# Autodesk Inventor assembly: ArmBase
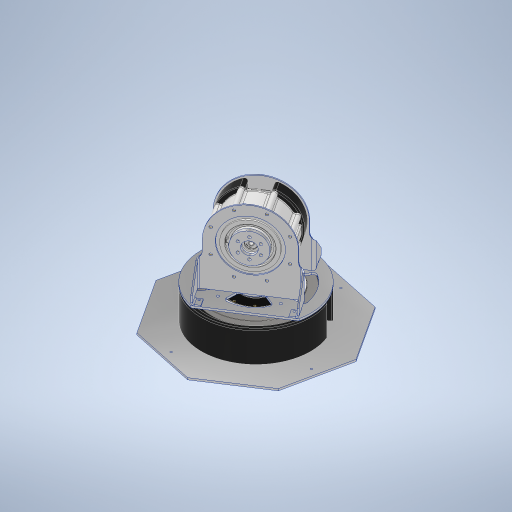
[picture p0: Inventor's stored thumbnail of the model, 512x512]
Saved by Autodesk Inventor 2024.3 (Build 283343010, 343A)
## iProperties
Created: 2025-05-20
Part Number: ArmBase
Document SubType Name: Assembly
Designer: kshau
Mass: 3061.84 g
Surface Area: 4858.08 cm^2
Volume: 1053.88 cm^3
Density: 2.9053 g/cm^3
Author: kshau
## Documents named in this file (16)
- C:\Users\kshau\Documents\inventor\Create_ViperX\Create_ViperX_ALOHA\Base_Component\ArmBase.iam
- C:\Users\kshau\Documents\inventor\Create_ViperX\Create_ViperX_ALOHA\Base_Component\base_parameter.ipt
- C:\Users\kshau\Documents\inventor\Create_ViperX\Create_ViperX_ALOHA\Actuator\RS02\RS02\RS02.iam
- C:\Users\kshau\Documents\inventor\Create_ViperX\Create_ViperX_ALOHA\BasicParts\TurnTable\TurnTable_140\TurnTable_140.iam
- C:\Users\kshau\Documents\inventor\Create_ViperX\Create_ViperX_ALOHA\Actuator\RS03\RS03\RS03.iam
- C:\Users\kshau\Documents\inventor\Create_ViperX\Create_ViperX_ALOHA\Base_Component\basefixplate1_forR3.ipt
- C:\Users\kshau\Documents\inventor\Create_ViperX\Create_ViperX_ALOHA\Base_Component\basefixpart_forR3.ipt
- C:\Users\kshau\Documents\inventor\Create_ViperX\Create_ViperX_ALOHA\Base_Component\basefixplate2_forR3.ipt
- C:\Users\kshau\Documents\inventor\Create_ViperX\Create_ViperX_ALOHA\Base_Component\servoplate_forR3.ipt
- C:\Users\kshau\Documents\inventor\Create_ViperX\Create_ViperX_ALOHA\Base_Component\baseplate_R2toR3.ipt
- C:\Users\kshau\Documents\inventor\Create_ViperX\Create_ViperX_ALOHA\Base_Component\basepart1_forR2.ipt
- C:\Users\kshau\Documents\inventor\Create_ViperX\Create_ViperX_ALOHA\Base_Component\basepart2_forR2.ipt
- C:\Users\kshau\Documents\inventor\Create_ViperX\Create_ViperX_ALOHA\NessesaryParts\ALSBF10-40-M4-N4\ALSBF10-40-M4-N4\ALSBF10-40-M4-N4.ipt
- C:\Users\kshau\Documents\inventor\Create_ViperX\Create_ViperX_ALOHA\Base_Component\Largebaseplate.ipt
- C:\Users\kshau\Documents\inventor\Create_ViperX\Create_ViperX_ALOHA\BasicParts\Bearing\NMB_RF2210X2HH\RF-2210X2HH.iam
- C:\Users\kshau\Documents\inventor\Create_ViperX\Create_ViperX_ALOHA\Base_Component\basespacer1.ipt
## Components (19 placed, 15 different names)
1. base_parameter:1
2. RS02:1 [sub-assembly] — メイト:1, 回転:15, 回転:16, 回転:17, メイト:2, 回転:29
3. TurnTable_140:1 [sub-assembly] — メイト:1, 回転:18, 回転:19, 回転:20, 回転:21, 回転:27, 回転:28
4. RS03:1 [sub-assembly] — 回転:3, 回転:4, 回転:5, 回転:6, 回転:9, 回転:10
5. basefixplate1_forR3:1 — 回転:3, 回転:4, 回転:26, フラッシュ:3
6. basefixpart_forR3:1 — 回転:5, 回転:6, 回転:11, 回転:12, メイト:5, メイト:6
7. basefixplate2_forR3:1 — 回転:11, 回転:12, 回転:25, フラッシュ:4
8. servoplate_forR3:1 — 回転:9, 回転:10
9. baseplate_R2toR3:1 — 回転:15, 回転:25, 回転:26, フラッシュ:3, フラッシュ:4, 回転:29, 回転:30, 回転:31
10. basepart1_forR2:1 — 回転:16, 回転:17, フラッシュ:1, フラッシュ:2, メイト:4, 回転:24
11. basepart2_forR2:1 — フラッシュ:1, メイト:2, メイト:3
12. ALSBF10-40-M4-N4:1 — 回転:18
13. ALSBF10-40-M4-N4:2 — 回転:19
14. ALSBF10-40-M4-N4:3 — 回転:20, 回転:23
15. ALSBF10-40-M4-N4:4 — 回転:21, 回転:22
16. basepart2_forR2:2 — フラッシュ:2, メイト:3, メイト:4
17. Largebaseplate:1 — 回転:22, 回転:23, 回転:24
18. RF-2210X2HH:1 [sub-assembly] — メイト:5, メイト:6
19. basespacer1:1 — 回転:27, 回転:28, 回転:30, 回転:31
## Relationships (35: RevoluteJoint 25, Mate 6, Flush 4)
- メイト:1 [Mate]: RS02:1 ↔ TurnTable_140:1
- 回転:3 [RevoluteJoint]: RS03:1 ↔ basefixplate1_forR3:1
- 回転:4 [RevoluteJoint]: RS03:1 ↔ basefixplate1_forR3:1
- 回転:5 [RevoluteJoint]: RS03:1 ↔ basefixpart_forR3:1
- 回転:6 [RevoluteJoint]: RS03:1 ↔ basefixpart_forR3:1
- 回転:9 [RevoluteJoint]: RS03:1 ↔ servoplate_forR3:1
- 回転:10 [RevoluteJoint]: RS03:1 ↔ servoplate_forR3:1
- 回転:11 [RevoluteJoint]: basefixpart_forR3:1 ↔ basefixplate2_forR3:1
- 回転:12 [RevoluteJoint]: basefixpart_forR3:1 ↔ basefixplate2_forR3:1
- 回転:15 [RevoluteJoint]: RS02:1 ↔ baseplate_R2toR3:1
- 回転:16 [RevoluteJoint]: RS02:1 ↔ basepart1_forR2:1
- 回転:17 [RevoluteJoint]: RS02:1 ↔ basepart1_forR2:1
- 回転:18 [RevoluteJoint]: TurnTable_140:1 ↔ ALSBF10-40-M4-N4:1
- 回転:19 [RevoluteJoint]: TurnTable_140:1 ↔ ALSBF10-40-M4-N4:2
- 回転:20 [RevoluteJoint]: TurnTable_140:1 ↔ ALSBF10-40-M4-N4:3
- 回転:21 [RevoluteJoint]: TurnTable_140:1 ↔ ALSBF10-40-M4-N4:4
- フラッシュ:1 [Flush]: basepart1_forR2:1 ↔ basepart2_forR2:1
- メイト:2 [Mate]: RS02:1 ↔ basepart2_forR2:1
- フラッシュ:2 [Flush]: basepart1_forR2:1 ↔ basepart2_forR2:2
- メイト:3 [Mate] (30 mm): basepart2_forR2:1 ↔ basepart2_forR2:2
- メイト:4 [Mate]: basepart1_forR2:1 ↔ basepart2_forR2:2
- 回転:22 [RevoluteJoint]: ALSBF10-40-M4-N4:4 ↔ Largebaseplate:1
- 回転:23 [RevoluteJoint]: ALSBF10-40-M4-N4:3 ↔ Largebaseplate:1
- 回転:24 [RevoluteJoint]: basepart1_forR2:1 ↔ Largebaseplate:1
- 回転:25 [RevoluteJoint]: basefixplate2_forR3:1 ↔ baseplate_R2toR3:1
- 回転:26 [RevoluteJoint]: basefixplate1_forR3:1 ↔ baseplate_R2toR3:1
- フラッシュ:3 [Flush]: basefixplate1_forR3:1 ↔ baseplate_R2toR3:1
- フラッシュ:4 [Flush]: basefixplate2_forR3:1 ↔ baseplate_R2toR3:1
- メイト:5 [Mate]: basefixpart_forR3:1 ↔ RF-2210X2HH:1
- メイト:6 [Mate]: basefixpart_forR3:1 ↔ RF-2210X2HH:1
- 回転:27 [RevoluteJoint]: TurnTable_140:1 ↔ basespacer1:1
- 回転:28 [RevoluteJoint]: TurnTable_140:1 ↔ basespacer1:1
- 回転:29 [RevoluteJoint]: RS02:1 ↔ baseplate_R2toR3:1
- 回転:30 [RevoluteJoint]: baseplate_R2toR3:1 ↔ basespacer1:1
- 回転:31 [RevoluteJoint]: baseplate_R2toR3:1 ↔ basespacer1:1
